# Autodesk Inventor assembly: PC104_EM-113 Assembly
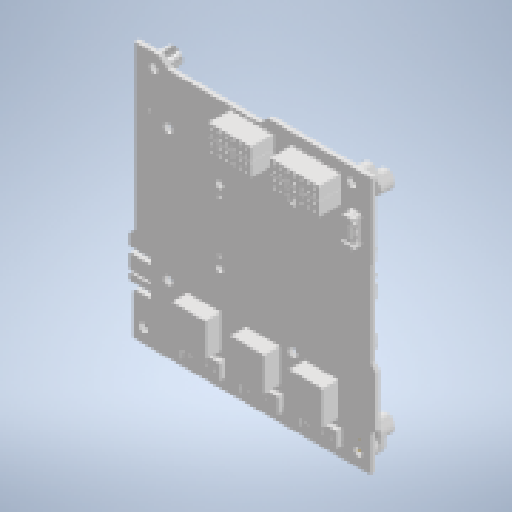
[picture p0: Inventor's stored thumbnail of the model, 512x512]
Saved by Autodesk Inventor 2024 (Build 280153000, 153)
## iProperties
Created: 2023-04-20
Part Number: PC104_EM-113 Assembly
Document SubType Name: Assembly
Designer: Owner
Author: Owner
## Documents named in this file (6)
- C:\Users\User\Documents\1UFrame\PC104_EM-113 Assembly.iam
- C:\Users\User\Documents\1UFrame\isispace-icepsv2-e-1_typeb.ipt
- C:\Users\User\Documents\1UFrame\PC104_EM-113 standoff_4.563.ipt
- C:\Users\User\Documents\1UFrame\PC104_EM-113 standoff_4.746.ipt
- C:\Users\User\Documents\1UFrame\PC104_EM-113 standoff_3.57.ipt
- C:\Users\User\Documents\1UFrame\PC104_EM-113 standoff_3.268.ipt
## Components (5 placed, 5 different names)
1. isispace-icepsv2-e-1_typeb:1 — Mate:14, Mate:16, Mate:17
2. PC104_EM-113 standoff_4.563:1
3. PC104_EM-113 standoff_4.746:1 — Mate:14
4. PC104_EM-113 standoff_3.57:1 — Mate:16, Mate:17
5. PC104_EM-113 standoff_3.268:1
## Relationships (3: Mate 3)
- Mate:14: isispace-icepsv2-e-1_typeb:1 ↔ PC104_EM-113 standoff_4.746:1
- Mate:16: isispace-icepsv2-e-1_typeb:1 ↔ PC104_EM-113 standoff_3.57:1
- Mate:17: isispace-icepsv2-e-1_typeb:1 ↔ PC104_EM-113 standoff_3.57:1
